# Autodesk Inventor assembly: ПД Модуль 100х100
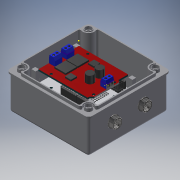
[picture p0: Inventor's stored thumbnail of the model, 180x180]
Saved by Autodesk Inventor 2019 (Build 230136000, 136)
## iProperties
Created: 2020-04-14
Part Number: ПД Модуль 100х100
Material: Типовые
Document SubType Name: Assembly
Designer: Surflay
Author: Surflay
## Documents named in this file (7)
- C:\Users\Surflay\Desktop\Университет\ПД\Модели\ПД Модуль 100х100.iam
- C:\Users\Surflay\Desktop\Университет\ПД\Модели\ПД Коробка 100х100х50.ipt
- C:\Users\Surflay\Desktop\Университет\ПД\RobotWheel\Arduino Uno with Sensor Shield\A_Arduino_Uno_Wifi_Shield.iam
- C:\Users\Surflay\Desktop\Университет\ПД\Модели\Monster_motor_Shield.ipt
- Troyka_Shield.ipt
- C:\Users\Surflay\Desktop\Университет\ПД\Модели\5-pin\5-pin.iam
- C:\Users\Surflay\Desktop\Университет\ПД\Модели\Каркас для плат.ipt
## Components (6 placed, 5 different names)
1. ПД Коробка 100х100х50:1 — Угол:1, Угол:4, Совмещение:2, Заподлицо:1, Совмещение:3, Угол:5, Угол:6, Заподлицо:2, Вставка:2, Угол:7, Вставка:3, Совмещение:7
2. A_Arduino_Uno_Wifi_Shield:1 [sub-assembly] — Угол:1, Угол:2, Угол:3, Вставка:1, Угол:4, Совмещение:2, Совмещение:4, Совмещение:5, Совмещение:6
3. Troyka_Shield:1 — Угол:2, Угол:3, Вставка:1, Совмещение:3
4. kls15-225-m12:1 [sub-assembly] — Угол:5, Угол:6, Вставка:2
5. kls15-225-m12:2 [sub-assembly] — Угол:7, Вставка:3
6. Каркас для плат:1 — Совмещение:4, Совмещение:5, Совмещение:6, Заподлицо:3, Совмещение:7
## Relationships (19: Angle 7, Mate 6, Insert 3, Flush 3)
- Угол:1 [Angle] (180 deg): ПД Коробка 100х100х50:1 ↔ A_Arduino_Uno_Wifi_Shield:1
- Угол:2 [Angle] (0 deg): A_Arduino_Uno_Wifi_Shield:1 ↔ Troyka_Shield:1
- Угол:3 [Angle] (90 deg): A_Arduino_Uno_Wifi_Shield:1 ↔ Troyka_Shield:1
- Вставка:1 [Insert] (-16 mm): A_Arduino_Uno_Wifi_Shield:1 ↔ Troyka_Shield:1
- Угол:4 [Angle] (0 deg): ПД Коробка 100х100х50:1 ↔ A_Arduino_Uno_Wifi_Shield:1
- Совмещение:2 [Mate] (23 mm): ПД Коробка 100х100х50:1 ↔ A_Arduino_Uno_Wifi_Shield:1
- Заподлицо:1 [Flush]: ПД Коробка 100х100х50:1
- Совмещение:3 [Mate] (10 mm): ПД Коробка 100х100х50:1 ↔ Troyka_Shield:1
- Угол:5 [Angle] (180 deg): ПД Коробка 100х100х50:1 ↔ kls15-225-m12:1
- Угол:6 [Angle] (180 deg): ПД Коробка 100х100х50:1 ↔ kls15-225-m12:1
- Заподлицо:2 [Flush]: ПД Коробка 100х100х50:1
- Вставка:2 [Insert] (-4 mm): ПД Коробка 100х100х50:1 ↔ kls15-225-m12:1
- Угол:7 [Angle] (180 deg): ПД Коробка 100х100х50:1 ↔ kls15-225-m12:2
- Вставка:3 [Insert]: ПД Коробка 100х100х50:1 ↔ kls15-225-m12:2
- Совмещение:4 [Mate]: A_Arduino_Uno_Wifi_Shield:1 ↔ Каркас для плат:1
- Совмещение:5 [Mate]: A_Arduino_Uno_Wifi_Shield:1 ↔ Каркас для плат:1
- Совмещение:6 [Mate]: A_Arduino_Uno_Wifi_Shield:1 ↔ Каркас для плат:1
- Заподлицо:3 [Flush]: Каркас для плат:1
- Совмещение:7 [Mate]: ПД Коробка 100х100х50:1 ↔ Каркас для плат:1
